# Autodesk Inventor assembly: 0401 ASY GBK wall shield Center 1
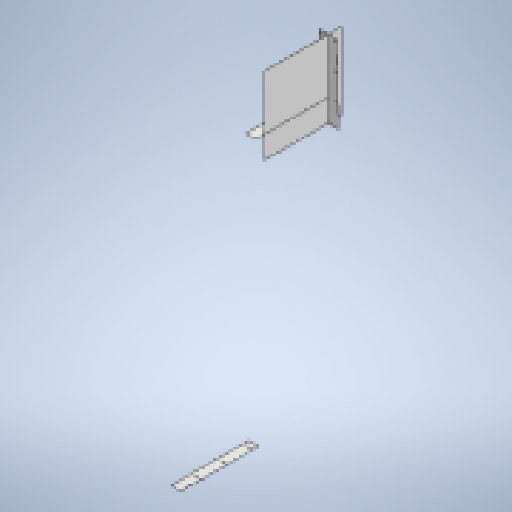
[picture p0: Inventor's stored thumbnail of the model, 512x512]
Saved by Autodesk Inventor 2026 (Build 300175000, 175)
## iProperties
Created: 2026-05-19
Part Number: 0401 ASY GBK wall shield Center 1
Document SubType Name: Assembly
Designer: admin
Author: admin
## Documents named in this file (6)
- C:\Users\pokla\Documents\Inventor\GBK-Gubkinskiy\0401 ASY GBK wall shield Center 1.iam
- C:\Users\pokla\Documents\Inventor\GBK-Gubkinskiy\0411 GBK Center main rib.ipt
- C:\Users\pokla\Documents\Inventor\GBK-Gubkinskiy\0413 GBK stringer C1.ipt
- C:\Users\pokla\Documents\Inventor\GBK-Gubkinskiy\01.1 GBK shield.ipt
- C:\Users\pokla\Documents\Inventor\GBK-Gubkinskiy\0414 GBK stringer C2.ipt
- C:\Users\pokla\Documents\Inventor\GBK-Gubkinskiy\0415 GBK stringer C3.ipt
## Components (6 placed, 5 different names)
1. 0411 GBK Center main rib:1 — Жесткий:1, Заподлицо:3, Совмещение:5, Заподлицо:4, Заподлицо:5, Жесткий:2, Жесткий:3
2. 0413 GBK stringer C1:1 — Жесткий:1
3. Part111:1 — Совмещение:1, Заподлицо:1, Совмещение:2, Заподлицо:2, Совмещение:4, Заподлицо:3, Совмещение:5, Заподлицо:5
4. 0411 GBK Center main rib:2 — Заподлицо:2, Совмещение:4, Заподлицо:4
5. 0414 GBK stringer C2:1 — Жесткий:2
6. 0415 GBK stringer C3:1 — Жесткий:3
## Relationships (12: Flush 5, Mate 4, WeldJoint 3)
- Жесткий:1 [WeldJoint] (4 mm): 0411 GBK Center main rib:1 ↔ 0413 GBK stringer C1:1
- Совмещение:1 [Mate]: Part111:1
- Заподлицо:1 [Flush]: Part111:1
- Совмещение:2 [Mate]: Part111:1
- Заподлицо:2 [Flush]: Part111:1 ↔ 0411 GBK Center main rib:2
- Совмещение:4 [Mate]: Part111:1 ↔ 0411 GBK Center main rib:2
- Заподлицо:3 [Flush]: 0411 GBK Center main rib:1 ↔ Part111:1
- Совмещение:5 [Mate]: 0411 GBK Center main rib:1 ↔ Part111:1
- Заподлицо:4 [Flush]: 0411 GBK Center main rib:1 ↔ 0411 GBK Center main rib:2
- Заподлицо:5 [Flush] (250 mm): 0411 GBK Center main rib:1 ↔ Part111:1
- Жесткий:2 [WeldJoint] (4 mm): 0411 GBK Center main rib:1 ↔ 0414 GBK stringer C2:1
- Жесткий:3 [WeldJoint] (4 mm): 0411 GBK Center main rib:1 ↔ 0415 GBK stringer C3:1
